# Autodesk Inventor assembly: PCBDiplomPCB
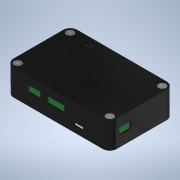
[picture p0: Inventor's stored thumbnail of the model, 180x180]
Saved by Autodesk Inventor 2022 (Build 260153000, 153)
## iProperties
Company: Open CASCADE
Created: 2022-01-03
Part Number: PCBDiplomPCB
Description: Open CASCADE Model
Document SubType Name: Assembly
Designer: user
Authority: Unknown
Mass: 40.7955 g
Surface Area: 403.085 cm^2
Volume: 26.6823 cm^3
Density: 1.52894 g/cm^3
Sending System: Open CASCADE 6.8
Preprocessor: Open CASCADE STEP processor 6.8
Title: Open CASCADE Shape Model
Author: Author
## Documents named in this file (41)
- C:\Study\Diplom\Altium\Diplom\Project Outputs for Diplom\Inventor\PCBDiplomPCB.iam
- C:\Study\Diplom\Altium\Diplom\Project Outputs for Diplom\Inventor\PCBBoard.iam
- C:\Study\Diplom\Altium\Diplom\Project Outputs for Diplom\Inventor\PCBZQ1.iam
- C:\Study\Diplom\Altium\Diplom\Project Outputs for Diplom\Inventor\PCBXS4.iam
- C:\Study\Diplom\Altium\Diplom\Project Outputs for Diplom\Inventor\PCBXS3.iam
- C:\Study\Diplom\Altium\Diplom\Project Outputs for Diplom\Inventor\PCBXS2.iam
- C:\Study\Diplom\Altium\Diplom\Project Outputs for Diplom\Inventor\PCBXS1.iam
- C:\Study\Diplom\Altium\Diplom\Project Outputs for Diplom\Inventor\PCBXP2.iam
- C:\Study\Diplom\Altium\Diplom\Project Outputs for Diplom\Inventor\PCBXP1.iam
- C:\Study\Diplom\Altium\Diplom\Project Outputs for Diplom\Inventor\PCBVT1.iam
- C:\Study\Diplom\Altium\Diplom\Project Outputs for Diplom\Inventor\PCBSB1.iam
- C:\Study\Diplom\Altium\Diplom\Project Outputs for Diplom\Inventor\PCBSA1.iam
- C:\Study\Diplom\Altium\Diplom\Project Outputs for Diplom\Inventor\PCBR7.iam
- C:\Study\Diplom\Altium\Diplom\Project Outputs for Diplom\Inventor\PCBR6.iam
- C:\Study\Diplom\Altium\Diplom\Project Outputs for Diplom\Inventor\PCBR5.iam
- C:\Study\Diplom\Altium\Diplom\Project Outputs for Diplom\Inventor\PCBR4.iam
- C:\Study\Diplom\Altium\Diplom\Project Outputs for Diplom\Inventor\PCBR3.iam
- C:\Study\Diplom\Altium\Diplom\Project Outputs for Diplom\Inventor\PCBR2.iam
- C:\Study\Diplom\Altium\Diplom\Project Outputs for Diplom\Inventor\PCBR1.iam
- C:\Study\Diplom\Altium\Diplom\Project Outputs for Diplom\Inventor\PCBL1.iam
- C:\Study\Diplom\Altium\Diplom\Project Outputs for Diplom\Inventor\PCBHL1.iam
- C:\Study\Diplom\Altium\Diplom\Project Outputs for Diplom\Inventor\PCBF1.iam
- C:\Study\Diplom\Altium\Diplom\Project Outputs for Diplom\Inventor\PCBDD1.iam
- C:\Study\Diplom\Altium\Diplom\Project Outputs for Diplom\Inventor\PCBDA1.iam
- C:\Study\Diplom\Altium\Diplom\Project Outputs for Diplom\Inventor\PCBC14.iam
- C:\Study\Diplom\Altium\Diplom\Project Outputs for Diplom\Inventor\PCBC13.iam
- C:\Study\Diplom\Altium\Diplom\Project Outputs for Diplom\Inventor\PCBC12.iam
- C:\Study\Diplom\Altium\Diplom\Project Outputs for Diplom\Inventor\PCBC11.iam
- C:\Study\Diplom\Altium\Diplom\Project Outputs for Diplom\Inventor\PCBC10.iam
- C:\Study\Diplom\Altium\Diplom\Project Outputs for Diplom\Inventor\PCBC9.iam
- C:\Study\Diplom\Altium\Diplom\Project Outputs for Diplom\Inventor\PCBC8.iam
- C:\Study\Diplom\Altium\Diplom\Project Outputs for Diplom\Inventor\PCBC7.iam
- C:\Study\Diplom\Altium\Diplom\Project Outputs for Diplom\Inventor\PCBC6.iam
- C:\Study\Diplom\Altium\Diplom\Project Outputs for Diplom\Inventor\PCBC5.iam
- C:\Study\Diplom\Altium\Diplom\Project Outputs for Diplom\Inventor\PCBC4.iam
- C:\Study\Diplom\Altium\Diplom\Project Outputs for Diplom\Inventor\PCBC3.iam
- C:\Study\Diplom\Altium\Diplom\Project Outputs for Diplom\Inventor\PCBC2.iam
- C:\Study\Diplom\Altium\Diplom\Project Outputs for Diplom\Inventor\PCBC1.iam
- C:\Study\Diplom\Altium\Diplom\Project Outputs for Diplom\Inventor\Основание.ipt
- C:\Study\Diplom\Altium\Diplom\Project Outputs for Diplom\Inventor\Крышка.ipt
- C:\Users\user\Documents\Inventor\Content Center Files\R2022\ru-RU\SFS 2977\SFS 2977 - M3 x 18.ipt
## Components (43 placed, 40 different names)
1. Board_2 [sub-assembly] — Вставка:1, Вставка:2
2. ZQ1_4 [sub-assembly]
3. XS4_6 [sub-assembly]
4. XS3_8 [sub-assembly]
5. XS2_10 [sub-assembly]
6. XS1_12 [sub-assembly]
7. XP2_16 [sub-assembly]
8. XP1_22 [sub-assembly]
9. VT1_24 [sub-assembly]
10. SB1_26 [sub-assembly]
11. SA1_29 [sub-assembly]
12. R7_31 [sub-assembly]
13. R6_33 [sub-assembly]
14. R5_35 [sub-assembly]
15. R4_37 [sub-assembly]
16. R3_39 [sub-assembly]
17. R2_41 [sub-assembly]
18. R1_43 [sub-assembly]
19. L1_48 [sub-assembly]
20. HL1_50 [sub-assembly]
21. F1_52 [sub-assembly]
22. DD1_54 [sub-assembly]
23. DA1_56 [sub-assembly]
24. C14_58 [sub-assembly]
25. C13_60 [sub-assembly]
26. C12_62 [sub-assembly]
27. C11_64 [sub-assembly]
28. C10_66 [sub-assembly]
29. C9_68 [sub-assembly]
30. C8_70 [sub-assembly]
31. C7_72 [sub-assembly]
32. C6_74 [sub-assembly]
33. C5_76 [sub-assembly]
34. C4_78 [sub-assembly]
35. C3_80 [sub-assembly]
36. C2_82 [sub-assembly]
37. C1_84 [sub-assembly]
38. Основание:1 — Вставка:1
39. Крышка:1 — Вставка:2, Совмещение:1, Совмещение:2, Совмещение:3, Совмещение:4
40. SFS 2977 M3 x 18:1 — Совмещение:1
41. SFS 2977 M3 x 18:2 — Совмещение:2
42. SFS 2977 M3 x 18:3 — Совмещение:3
43. SFS 2977 M3 x 18:4 — Совмещение:4
## Relationships (6: Mate 4, Insert 2)
- Вставка:1 [Insert]: Board_2 ↔ Основание:1
- Вставка:2 [Insert]: Board_2 ↔ Крышка:1
- Совмещение:1 [Mate]: Крышка:1 ↔ SFS 2977 M3 x 18:1
- Совмещение:2 [Mate]: Крышка:1 ↔ SFS 2977 M3 x 18:2
- Совмещение:3 [Mate]: Крышка:1 ↔ SFS 2977 M3 x 18:3
- Совмещение:4 [Mate]: Крышка:1 ↔ SFS 2977 M3 x 18:4
